# Autodesk Inventor assembly: AssemblyYijie
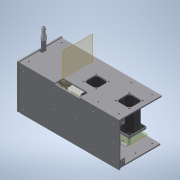
[picture p0: Inventor's stored thumbnail of the model, 180x180]
Saved by Autodesk Inventor 2020 (Build 240168000, 168)
## iProperties
Created: 2021-03-03
Part Number: AssemblyYijie
Document SubType Name: Assembly
Designer: LuoYi
Author: LuoYi
## Documents named in this file (23)
- C:\Users\UCLA\Desktop\VI_toYijie\VI_inventor\AssemblyYijie.iam
- C:\Users\UCLA\Desktop\VI_toYijie\VI_inventor\VirtualImpavtor.iam
- C:\Users\UCLA\Desktop\VI_toYijie\VI_inventor\AWM3100.ipt
- C:\Users\UCLA\Desktop\VI_toYijie\VI_inventor\tubeThinCurve.ipt
- C:\Users\UCLA\Desktop\VI_toYijie\VI_inventor\middleBase.ipt
- C:\Users\UCLA\Desktop\VI_toYijie\VI_inventor\fanConnector.ipt
- C:\Users\UCLA\Desktop\VI_toYijie\VI_inventor\fan.ipt
- C:\Users\UCLA\Desktop\VI_toYijie\VI_inventor\ySplitter.ipt
- C:\Users\UCLA\Desktop\VI_toYijie\VI_inventor\flowMeter.ipt
- C:\Users\UCLA\Desktop\VI_toYijie\VI_inventor\lowerBase.ipt
- C:\Users\UCLA\Desktop\VI_toYijie\VI_inventor\sensorBoard.ipt
- C:\Users\UCLA\Desktop\VI_toYijie\VI_inventor\sideWallRight.ipt
- C:\Users\UCLA\Desktop\VI_toYijie\VI_inventor\twoSideHold.ipt
- C:\Users\UCLA\Desktop\VI_toYijie\VI_inventor\fanCounterRotateConnector.ipt
- C:\Users\UCLA\Desktop\VI_toYijie\VI_inventor\fanCounterRotating.ipt
- C:\Users\UCLA\Desktop\VI_toYijie\VI_inventor\post.ipt
- C:\Users\UCLA\Desktop\VI_toYijie\VI_inventor\threeSideHold.ipt
- C:\Users\UCLA\Desktop\VI_toYijie\VI_inventor\sideWallTop .ipt
- C:\Users\UCLA\Desktop\VI_toYijie\VI_inventor\sideWallFront.0002.ipt
- C:\Users\UCLA\Desktop\VI_toYijie\VI_inventor\sideWallBack.ipt
- C:\Users\UCLA\Desktop\VI_toYijie\VI_inventor\sideWallLeft.ipt
- C:\Users\UCLA\Desktop\VI_toYijie\VI_inventor\tube20mm.ipt
- C:\Users\UCLA\Desktop\VI_toYijie\VI_inventor\laserCapV3.ipt
## Components (41 placed, 22 different names)
1. sideWallRight:1 — Mate:31, Mate:37, Flush:4, Mate:52, Mate:59, Mate:61, Flush:6, Mate:72, Mate:73, Mate:76, Mate:78, Mate:81, Flush:8
2. sideWallFront.0002:1 — Mate:83, Mate:84, Mate:92, Mate:111, Mate:113, Mate:115
3. sideWallTop :1 — Mate:62, Flush:6, Mate:63, Mate:65, Mate:66, Mate:67, Mate:69, Mate:70, Mate:75, Mate:79
4. sideWallLeft:1 — Mate:101, Mate:102, Mate:110, Mate:112
5. lowerBase:1 — Flush:2, Mate:20, Mate:21, Mate:30, Mate:31, Flush:4, Mate:41, Angle:1, Mate:54, Mate:55, Mate:71, Mate:74, Mate:77, Mate:93, Mate:94, Mate:114
6. threeSideHold:1 — Mate:52, Mate:113, Mate:114
7. sideWallBack:1 — Mate:85, Mate:86, Mate:87, Mate:88, Mate:89, Mate:95, Mate:98, Flush:9
8. VirtualImpavtor:1 [sub-assembly] — Mate:1, Mate:2, Mate:3, Mate:4, Mate:5, Mate:8, Mate:16, Mate:17, Mate:18, Mate:22, Mate:24, Mate:90, Mate:91, Mate:106, Flush:10, Mate:116, Mate:117, Mate:118
9. AWM3100:1 — Mate:4, Mate:5, Mate:6, Mate:9, Mate:107
10. tubeThinCurve:1 — Mate:6, Mate:11
11. middleBase:1 — Mate:8, Mate:9, Flush:2, Mate:22, Angle:1, Mate:42, Mate:43, Mate:44, Mate:45, Mate:46, Mate:47, Mate:48, Mate:49
12. fanConnector:1 — Mate:11, Mate:68, Flush:7
13. fan:1 — Mate:65, Mate:66, Mate:67, Mate:68, Flush:7
14. ySplitter:1 — Mate:16, Mate:17, Mate:18, Mate:19, Mate:20, Mate:21
15. flowMeter:1 — Mate:19, Mate:41, Mate:108, Mate:109
16. sensorBoard:1 — Mate:24, Mate:90, Mate:91, Mate:102
17. tubeThinCurve:2 — Mate:30, Mate:37
18. fanCounterRotateConnector:1 — Mate:38, Mate:39, Mate:40
19. fanCounterRotating:1 — Mate:38, Mate:39, Mate:40, Mate:69, Mate:70
20. post:1 — Mate:46, Mate:47
21. post:2 — Mate:48, Mate:49
22. post:3 — Mate:44, Mate:45
23. post:4 — Mate:42, Mate:43
24. twoSideHold:2 — Mate:54, Mate:55, Mate:115
25. twoSideHold:3 — Mate:59, Mate:81, Flush:8
26. threeSideHold:2 — Mate:61, Mate:62, Mate:63, Mate:83, Mate:84
27. twoSideHold:4 — Mate:71, Mate:72
28. threeSideHold:3 — Mate:73, Mate:74
29. threeSideHold:4 — Mate:75, Mate:76, Mate:85, Mate:89
30. twoSideHold:5 — Mate:77, Mate:87
31. twoSideHold:6 — Mate:79, Mate:88
32. twoSideHold:7 — Mate:78, Mate:86
33. threeSideHold:5 — Mate:92, Mate:93, Mate:110
34. threeSideHold:6 — Mate:94, Mate:95
35. twoSideHold:8 — Mate:98, Flush:9, Mate:101
36. tube20mm:1 — Mate:106
37. tube20mm:2 — Mate:107
38. tube20mm:3 — Mate:109
39. tube20mm:4 — Mate:108
40. threeSideHold:7 — Mate:111, Mate:112
41. laserCapV3:1 — Mate:116, Mate:117, Mate:118
## Relationships (92: Mate 84, Flush 7, Angle 1)
- Mate:1: VirtualImpavtor:1
- Mate:2: VirtualImpavtor:1
- Mate:3: VirtualImpavtor:1
- Mate:4: VirtualImpavtor:1 ↔ AWM3100:1
- Mate:5 (10 mm): VirtualImpavtor:1 ↔ AWM3100:1
- Mate:6: AWM3100:1 ↔ tubeThinCurve:1
- Mate:8 (30 mm): VirtualImpavtor:1 ↔ middleBase:1
- Mate:9: AWM3100:1 ↔ middleBase:1
- Mate:11: tubeThinCurve:1 ↔ fanConnector:1
- Mate:16: VirtualImpavtor:1 ↔ ySplitter:1
- Mate:17: VirtualImpavtor:1 ↔ ySplitter:1
- Mate:18 (-3 mm): VirtualImpavtor:1 ↔ ySplitter:1
- Mate:19: ySplitter:1 ↔ flowMeter:1
- Flush:2: lowerBase:1 ↔ middleBase:1
- Mate:20: lowerBase:1 ↔ ySplitter:1
- Mate:21: lowerBase:1 ↔ ySplitter:1
- Mate:22: VirtualImpavtor:1 ↔ middleBase:1
- Mate:24: VirtualImpavtor:1 ↔ sensorBoard:1
- Mate:30: lowerBase:1 ↔ tubeThinCurve:2
- Mate:31: sideWallRight:1 ↔ lowerBase:1
- Mate:37: sideWallRight:1 ↔ tubeThinCurve:2
- Mate:38 (-5 mm): fanCounterRotateConnector:1 ↔ fanCounterRotating:1
- Mate:39: fanCounterRotateConnector:1 ↔ fanCounterRotating:1
- Mate:40: fanCounterRotateConnector:1 ↔ fanCounterRotating:1
- Flush:4: sideWallRight:1 ↔ lowerBase:1
- Mate:41: lowerBase:1 ↔ flowMeter:1
- Angle:1 (0 deg): lowerBase:1 ↔ middleBase:1
- Mate:42: middleBase:1 ↔ post:4
- Mate:43: middleBase:1 ↔ post:4
- Mate:44: middleBase:1 ↔ post:3
- Mate:45: middleBase:1 ↔ post:3
- Mate:46: middleBase:1 ↔ post:1
- Mate:47: middleBase:1 ↔ post:1
- Mate:48: middleBase:1 ↔ post:2
- Mate:49: middleBase:1 ↔ post:2
- Mate:52: sideWallRight:1 ↔ threeSideHold:1
- Mate:54: lowerBase:1 ↔ twoSideHold:2
- Mate:55: lowerBase:1 ↔ twoSideHold:2
- Mate:59: sideWallRight:1 ↔ twoSideHold:3
- Mate:61: sideWallRight:1 ↔ threeSideHold:2
- Mate:62: sideWallTop :1 ↔ threeSideHold:2
- Flush:6: sideWallRight:1 ↔ sideWallTop :1
- Mate:63: sideWallTop :1 ↔ threeSideHold:2
- Mate:65: sideWallTop :1 ↔ fan:1
- Mate:66: sideWallTop :1 ↔ fan:1
- Mate:67: sideWallTop :1 ↔ fan:1
- Mate:68: fanConnector:1 ↔ fan:1
- Flush:7: fanConnector:1 ↔ fan:1
- Mate:69: sideWallTop :1 ↔ fanCounterRotating:1
- Mate:70: sideWallTop :1 ↔ fanCounterRotating:1
- Mate:71: lowerBase:1 ↔ twoSideHold:4
- Mate:72: sideWallRight:1 ↔ twoSideHold:4
- Mate:73: sideWallRight:1 ↔ threeSideHold:3
- Mate:74: lowerBase:1 ↔ threeSideHold:3
- Mate:75: sideWallTop :1 ↔ threeSideHold:4
- Mate:76: sideWallRight:1 ↔ threeSideHold:4
- Mate:77: lowerBase:1 ↔ twoSideHold:5
- Mate:78: sideWallRight:1 ↔ twoSideHold:7
- Mate:79: sideWallTop :1 ↔ twoSideHold:6
- Mate:81: sideWallRight:1 ↔ twoSideHold:3
- Flush:8: sideWallRight:1 ↔ twoSideHold:3
- Mate:83: sideWallFront.0002:1 ↔ threeSideHold:2
- Mate:84: sideWallFront.0002:1 ↔ threeSideHold:2
- Mate:85: sideWallBack:1 ↔ threeSideHold:4
- Mate:86: sideWallBack:1 ↔ twoSideHold:7
- Mate:87: sideWallBack:1 ↔ twoSideHold:5
- Mate:88: sideWallBack:1 ↔ twoSideHold:6
- Mate:89: sideWallBack:1 ↔ threeSideHold:4
- Mate:90: VirtualImpavtor:1 ↔ sensorBoard:1
- Mate:91: VirtualImpavtor:1 ↔ sensorBoard:1
- Mate:92: sideWallFront.0002:1 ↔ threeSideHold:5
- Mate:93: lowerBase:1 ↔ threeSideHold:5
- Mate:94: lowerBase:1 ↔ threeSideHold:6
- Mate:95: sideWallBack:1 ↔ threeSideHold:6
- Mate:98: sideWallBack:1 ↔ twoSideHold:8
- Flush:9: sideWallBack:1 ↔ twoSideHold:8
- Mate:101: sideWallLeft:1 ↔ twoSideHold:8
- Mate:102: sideWallLeft:1 ↔ sensorBoard:1
- Mate:106: VirtualImpavtor:1 ↔ tube20mm:1
- Mate:107: AWM3100:1 ↔ tube20mm:2
- Mate:108: flowMeter:1 ↔ tube20mm:4
- Mate:109: flowMeter:1 ↔ tube20mm:3
- Mate:110: sideWallLeft:1 ↔ threeSideHold:5
- Mate:111: sideWallFront.0002:1 ↔ threeSideHold:7
- Mate:112: sideWallLeft:1 ↔ threeSideHold:7
- Mate:113: sideWallFront.0002:1 ↔ threeSideHold:1
- Mate:114: lowerBase:1 ↔ threeSideHold:1
- Mate:115: sideWallFront.0002:1 ↔ twoSideHold:2
- Flush:10 (80 mm): VirtualImpavtor:1
- Mate:116: VirtualImpavtor:1 ↔ laserCapV3:1
- Mate:117: VirtualImpavtor:1 ↔ laserCapV3:1
- Mate:118: VirtualImpavtor:1 ↔ laserCapV3:1
